# Autodesk Inventor assembly: Rear B2
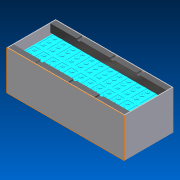
[picture p0: Inventor's stored thumbnail of the model, 180x180]
Saved by Autodesk Inventor 2012 (Build 160160000, 160)
## iProperties
Created: 2012-07-06
Part Number: Rear B2
Document SubType Name: Assembly
Designer: Hemant
Author: Hemant
## Documents named in this file (4)
- C:\Users\Hemant\Documents\Battery Boxes\BB REAR B\Rear B2.iam
- C:\Users\Hemant\Documents\Battery Boxes\BB REAR B\super large Battery Box Pastic 4.ipt
- C:\Users\Hemant\Documents\Battery Boxes\Batteries\CALB100AH final.ipt
- C:\Users\Hemant\Documents\Battery Boxes\BB REAR B\SPACER REAR B 1.ipt
## Components (27 placed, 3 different names)
1. super large Battery Box Pastic 4:1 — Mate:2, Mate:3, Mate:4, Mate:6, Mate:7
2. SPACER REAR B 1:1 — Mate:5, Mate:6, Mate:7
3. SPACER REAR B 1:2
4. CALB100AH final:1 — Mate:4
5. CALB100AH final:2 — Mate:2
6. CALB100AH final:3
7. CALB100AH final:4 — Mate:3
8. CALB100AH final:5
9. CALB100AH final:6
10. CALB100AH final:7
11. CALB100AH final:8 — Mate:5
12. CALB100AH final:9
13. CALB100AH final:10
14. CALB100AH final:11
15. CALB100AH final:12
16. CALB100AH final:13
17. CALB100AH final:14
18. CALB100AH final:15
19. CALB100AH final:16
20. CALB100AH final:17
21. CALB100AH final:18
22. CALB100AH final:19
23. CALB100AH final:20
24. CALB100AH final:21
25. CALB100AH final:22
26. CALB100AH final:23
27. CALB100AH final:24
## Component patterns: (12 elements), (2 elements, first: SPACER REAR B 1:1), (2 elements, first: CALB100AH final:1), Component Pattern 1:2 (2 elements), Component Pattern 1:3 (2 elements), Component Pattern 1:4 (2 elements), Component Pattern 1:5 (2 elements), Component Pattern 1:6 (2 elements), Component Pattern 1:7 (2 elements), Component Pattern 1:8 (2 elements), Component Pattern 1:9 (2 elements), Component Pattern 1:10 (2 elements), Component Pattern 1:11 (2 elements), Component Pattern 1:12 (2 elements)
## Relationships (6: Mate 6)
- Mate:2: super large Battery Box Pastic 4:1 ↔ CALB100AH final:2
- Mate:3 (25.4 mm): super large Battery Box Pastic 4:1 ↔ CALB100AH final:4
- Mate:4 (15.24 mm): super large Battery Box Pastic 4:1 ↔ CALB100AH final:1
- Mate:5: SPACER REAR B 1:1 ↔ CALB100AH final:8
- Mate:6: super large Battery Box Pastic 4:1 ↔ SPACER REAR B 1:1
- Mate:7: super large Battery Box Pastic 4:1 ↔ SPACER REAR B 1:1
